# Autodesk Inventor assembly: WheelAssembly
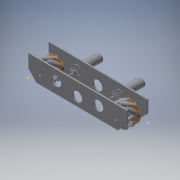
[picture p0: Inventor's stored thumbnail of the model, 180x180]
Saved by Autodesk Inventor 2017 (Build 210142000, 142)
## iProperties
Created: 2016-09-10
Part Number: WheelAssembly
Document SubType Name: Assembly
Designer: RoboticsUser
Author: RoboticsUser
## Documents named in this file (9)
- C:\Robotics\CAD\2016-17_CAD\WheelAssemble2.0.iam
- C:\Robotics\CAD\COTSParts\Actobotics\545 parts\545556.ipt
- C:\Robotics\CAD\COTSParts\Actobotics\615 parts\615102.ipt
- C:\Robotics\CAD\COTSParts\Actobotics\634 parts\634080.ipt
- C:\Robotics\CAD\COTSParts\Motors\Andymark 2964  NeveRest 40 Motor.ipt
- C:\Robotics\CAD\COTSParts\Tetrix\tetrix-motor-mounts-1.snapshot.1\Tetrex 2pc motor mount.ipt
- C:\Robotics\CAD\COTSParts\Actobotics\545 parts\545456.ipt
- C:\Robotics\CAD\COTSParts\Wheels\AndyMark Mecanum Wheels\100mm Aluminum Mecanum wheels.ipt
- C:\Robotics\CAD\2016-17_CAD\DrainTrainPlate2.0.iam
## Components (24 placed, 8 different names)
1. 545556:2 — Mate:10, Mate:13, Mate:47
2. 615102:4 — Mate:35, Mate:36, Mate:37, Flush:4
3. 634080:2 — Mate:10, Mate:12, Mate:26, Mate:32, Mate:45, Mate:52, Mate:56
4. 545556:6 — Insert:83, Mate:46
5. 615102:5 — Mate:2, Flush:3, Mate:44, Mate:46
6. 634080:3 — Mate:28, Mate:30, Mate:44, Mate:50, Mate:53, Mate:55, Mate:60, Flush:6
7. Andymark 2964  NeveRest 40 Motor:2 — Mate:39, Mate:41, Mate:42, Mate:43, Mate:57
8. 545556:8 — Mate:2, Mate:4, Mate:43
9. 545556:9 — Mate:37, Mate:38
10. Andymark 2964  NeveRest 40 Motor:3 — Mate:34, Mate:35, Mate:36, Mate:38, Mate:58, Flush:5
11. Tetrex 2pc motor mount:1 — Mate:39
12. Tetrex 2pc motor mount:2 — Mate:34, Mate:51
13. 545456:1 — Mate:12, Mate:13, Insert:89
14. 545456:3 — Insert:83, Insert:88
15. 615102:6 — Mate:4, Mate:41, Mate:42, Flush:3
16. 615102:7 — Flush:4, Mate:45, Mate:47
17. 100mm Aluminum Mecanum wheels:1 — Insert:88, Mate:27, Mate:50
18. 100mm Aluminum Mecanum wheels:2 — Insert:89, Mate:25
19. 545456:4 — Mate:25, Mate:26, Mate:31
20. 545456:5 — Mate:27, Mate:28, Mate:29
21. 545556:12 — Mate:29, Mate:30, Mate:54
22. 545556:13 — Mate:31, Mate:32, Mate:59
23. DrainTrainPlate2.0:1 [sub-assembly] — Mate:54, Mate:55, Mate:56, Mate:59, Mate:60, Flush:6
24. DrainTrainPlate2.0:2 [sub-assembly] — Mate:51, Mate:52, Mate:53, Mate:57, Mate:58, Flush:5
## Relationships (44: Mate 37, Flush 4, Insert 3)
- Insert:83: 545556:6 ↔ 545456:3
- Mate:2: 615102:5 ↔ 545556:8
- Mate:4: 545556:8 ↔ 615102:6
- Mate:10: 545556:2 ↔ 634080:2
- Mate:12: 634080:2 ↔ 545456:1
- Mate:13: 545556:2 ↔ 545456:1
- Insert:88: 545456:3 ↔ 100mm Aluminum Mecanum wheels:1
- Insert:89: 545456:1 ↔ 100mm Aluminum Mecanum wheels:2
- Mate:25: 100mm Aluminum Mecanum wheels:2 ↔ 545456:4
- Mate:26: 634080:2 ↔ 545456:4
- Mate:27: 100mm Aluminum Mecanum wheels:1 ↔ 545456:5
- Mate:28: 634080:3 ↔ 545456:5
- Mate:29: 545456:5 ↔ 545556:12
- Mate:30: 634080:3 ↔ 545556:12
- Mate:31: 545456:4 ↔ 545556:13
- Mate:32: 634080:2 ↔ 545556:13
- Mate:34: Andymark 2964  NeveRest 40 Motor:3 ↔ Tetrex 2pc motor mount:2
- Mate:35: 615102:4 ↔ Andymark 2964  NeveRest 40 Motor:3
- Mate:36: 615102:4 ↔ Andymark 2964  NeveRest 40 Motor:3
- Mate:37: 615102:4 ↔ 545556:9
- Mate:38: 545556:9 ↔ Andymark 2964  NeveRest 40 Motor:3
- Mate:39: Andymark 2964  NeveRest 40 Motor:2 ↔ Tetrex 2pc motor mount:1
- Mate:41: Andymark 2964  NeveRest 40 Motor:2 ↔ 615102:6
- Mate:42: Andymark 2964  NeveRest 40 Motor:2 ↔ 615102:6
- Mate:43: Andymark 2964  NeveRest 40 Motor:2 ↔ 545556:8
- Flush:3: 615102:5 ↔ 615102:6
- Mate:44: 615102:5 ↔ 634080:3
- Flush:4: 615102:4 ↔ 615102:7
- Mate:45: 634080:2 ↔ 615102:7
- Mate:46: 545556:6 ↔ 615102:5
- Mate:47: 545556:2 ↔ 615102:7
- Mate:50: 634080:3 ↔ 100mm Aluminum Mecanum wheels:1
- Mate:51: Tetrex 2pc motor mount:2 ↔ DrainTrainPlate2.0:2
- Mate:52: 634080:2 ↔ DrainTrainPlate2.0:2
- Mate:53: 634080:3 ↔ DrainTrainPlate2.0:2
- Mate:54: 545556:12 ↔ DrainTrainPlate2.0:1
- Mate:55: 634080:3 ↔ DrainTrainPlate2.0:1
- Mate:56: 634080:2 ↔ DrainTrainPlate2.0:1
- Mate:57: Andymark 2964  NeveRest 40 Motor:2 ↔ DrainTrainPlate2.0:2
- Mate:58: Andymark 2964  NeveRest 40 Motor:3 ↔ DrainTrainPlate2.0:2
- Flush:5: Andymark 2964  NeveRest 40 Motor:3 ↔ DrainTrainPlate2.0:2
- Mate:59: 545556:13 ↔ DrainTrainPlate2.0:1
- Mate:60: 634080:3 ↔ DrainTrainPlate2.0:1
- Flush:6: 634080:3 ↔ DrainTrainPlate2.0:1
